# Autodesk Inventor assembly: Blog Assembly
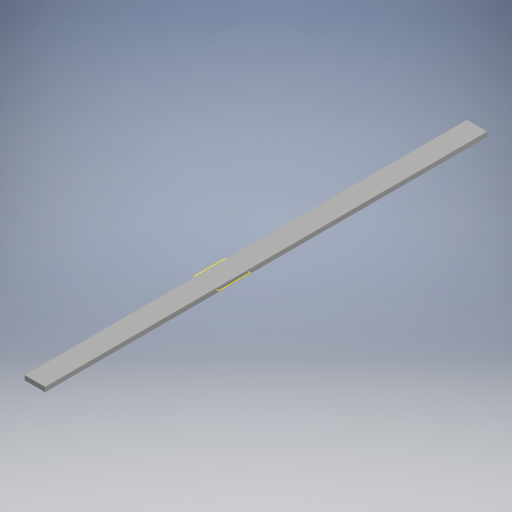
[picture p0: Inventor's stored thumbnail of the model, 512x512]
Saved by Autodesk Inventor 2024.2 (Build 282272000, 272)
## iProperties
Created: 2024-04-19
Part Number: Blog Assembly
Document SubType Name: Assembly
Designer: TiffanyHayden
FAMILY: ATQ
GATE LOCATION: 25'-0"
HEIGHT: 10'-0"
OAL: 65'-0"
Author: TiffanyHayden
## Documents named in this file (4)
- C:\Blog\Blog Assembly.iam
- C:\Blog\Assets\ATQ-36-120-N.ipt
- C:\Blog\Assets\ATQ-36-60-B.ipt
- C:\Blog\Assets\ATQ-36-60-N.ipt
## Components (9 placed, 5 different names)
1. GATE — Flush:10, Flush:11, Flush:12, Flush:16
2. COMP OUT — Flush:13, Flush:14, Flush:15, Flush:17
3. COMP IN — Flush:7, Flush:8, Flush:9
4. ATQ-36-120-N:5
5. ATQ-36-120-N:12
6. COMP GATE — Flush:18, Flush:19, Flush:20
7. ATQ-36-120-N:8
8. ATQ-36-120-N:9
9. ATQ-36-120-N:10
## Component patterns: PAT IN (3 elements), PAT OUT (4 elements)
## Relationships (20: Flush 20)
- Flush:1
- Flush:2 (19812 mm)
- Flush:3
- Flush:4
- Flush:5 (-3048 mm)
- Flush:6 (7620 mm)
- Flush:7: COMP IN
- Flush:8: COMP IN
- Flush:9: COMP IN
- Flush:10: GATE
- Flush:11: GATE
- Flush:12: GATE
- Flush:13: COMP OUT
- Flush:14: COMP OUT
- Flush:15: COMP OUT
- Flush:16: GATE
- Flush:17: COMP OUT
- Flush:18: COMP GATE
- Flush:19: COMP GATE
- Flush:20: COMP GATE
## Named parameters: OAL = 19812 mm, GATE_LOCATION = 7620 mm, HEIGHT = 3048 mm, PAT_IN_QTY = 3, PAT_OUT_QTY = 4, PAT_IN_OFFSET = 3048 mm, PAT_OUT_OFFSET = 3048 mm
